# Autodesk Inventor assembly: Assembly1
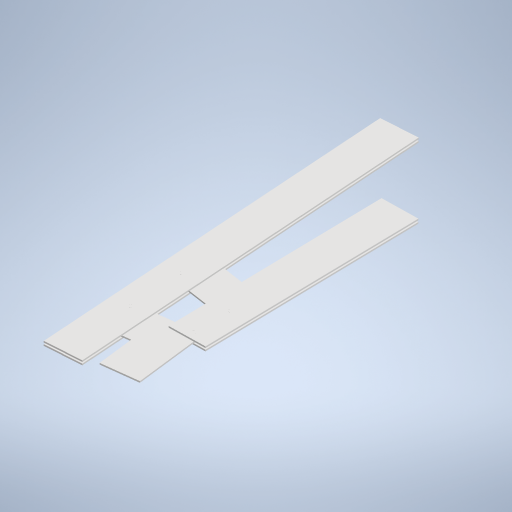
[picture p0: Inventor's stored thumbnail of the model, 512x512]
Saved by Autodesk Inventor 2023 (Build 270158000, 158)
## iProperties
Created: 2022-11-06
Part Number: Assembly1
Document SubType Name: Assembly
Designer: SAMJ
Author: SAMJ
## Documents named in this file (6)
- D:\Desktop\Pendientes\Robotica\ProyectoRobotica\ModeloGripperFinal\Assembly1.iam
- D:\Desktop\Pendientes\Robotica\ProyectoRobotica\ModeloGripperFinal\Axis.ipt
- D:\Desktop\Pendientes\Robotica\ProyectoRobotica\ModeloGripperFinal\H.ipt
- D:\Desktop\Pendientes\Robotica\ProyectoRobotica\ModeloGripperFinal\Ldw.ipt
- D:\Desktop\Pendientes\Robotica\ProyectoRobotica\ModeloGripperFinal\Lup.ipt
- D:\Desktop\Pendientes\Robotica\ProyectoRobotica\ModeloGripperFinal\Pinz.ipt
## Components (10 placed, 5 different names)
1. Axis:1 — Insert:4, Insert:5, Insert:11
2. H:1 — Insert:3, Insert:4
3. Ldw:1 — Insert:5, Insert:7
4. Lup:1 — Insert:1, Insert:2
5. Axis:2 — Insert:2, Insert:6, Insert:10
6. Axis:3 — Insert:1, Insert:3, Insert:9
7. Pinz:1 — Insert:6, Insert:8
8. Axis:4 — Insert:7, Insert:8, Insert:12
9. Ldw:2 — Insert:11, Insert:12
10. Lup:2 — Insert:9, Insert:10
## Relationships (12: Insert 12)
- Insert:1: Lup:1 ↔ Axis:3
- Insert:2: Lup:1 ↔ Axis:2
- Insert:3 (-2 mm): H:1 ↔ Axis:3
- Insert:4 (-2 mm): Axis:1 ↔ H:1
- Insert:5: Axis:1 ↔ Ldw:1
- Insert:6 (2 mm): Axis:2 ↔ Pinz:1
- Insert:7: Ldw:1 ↔ Axis:4
- Insert:8 (2 mm): Pinz:1 ↔ Axis:4
- Insert:9: Axis:3 ↔ Lup:2
- Insert:10: Axis:2 ↔ Lup:2
- Insert:11: Axis:1 ↔ Ldw:2
- Insert:12: Axis:4 ↔ Ldw:2
